# Autodesk Inventor assembly: Robot arm 01
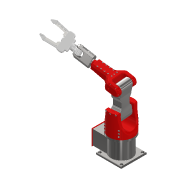
[picture p0: Inventor's stored thumbnail of the model, 180x180]
Saved by Autodesk Inventor 2020.3 (Build 243373010, 373A)
## iProperties
Created: 2021-04-17
Part Number: Robot arm 01
Document SubType Name: Assembly
Designer: marti
Mass: 362095 g
Surface Area: 35809.9 cm^2
Volume: 47437.3 cm^3
Density: 7.63313 g/cm^3
Author: marti
## Documents named in this file (30)
- C:\Users\marti\Documents\Inventor\RobotManipulateArm\17.4.2021 - Complete new IDEA\Robot arm 01.iam
- C:\Users\marti\Documents\Inventor\RobotManipulateArm\17.4.2021 - Complete new IDEA\Cover of robot - base upper part 02.ipt
- C:\Users\marti\Documents\Inventor\RobotManipulateArm\17.4.2021 - Complete new IDEA\Ground base of robot.ipt
- C:\Users\marti\Documents\Inventor\RobotManipulateArm\17.4.2021 - Complete new IDEA\base for robot 1\Base for robot 2.ipt
- C:\Users\marti\Documents\Inventor\RobotManipulateArm\17.4.2021 - Complete new IDEA\Servomotor_1.iam
- C:\Users\marti\Documents\Inventor\RobotManipulateArm\17.4.2021 - Complete new IDEA\Robot arm part 01.ipt
- C:\Users\marti\Documents\Inventor\RobotManipulateArm\17.4.2021 - Complete new IDEA\Head of robot arrm.ipt
- C:\Users\marti\Documents\Inventor\RobotManipulateArm\17.4.2021 - Complete new IDEA\Cover of robot base L.ipt
- C:\Users\marti\Documents\Inventor\Content Center Files\R2020\en-US\ISO 4762(1)\DIN EN ISO 4762 - M14 x 30.ipt
- C:\Users\marti\Documents\Inventor\RobotManipulateArm\17.4.2021 - Complete new IDEA\Cover of robot base R.ipt
- C:\Users\marti\Documents\Inventor\RobotManipulateArm\17.4.2021 - Complete new IDEA\Cover part of robot arm.ipt
- C:\Users\marti\Documents\Inventor\Content Center Files\R2020\en-US\ISO 4762(1)\DIN EN ISO 4762 - M10 x 25.ipt
- C:\Users\marti\Documents\Inventor\Content Center Files\R2020\en-US\ISO 4762(1)\DIN EN ISO 4762 - M12 x 25.ipt
- C:\Users\marti\Documents\Inventor\RobotManipulateArm\17.4.2021 - Complete new IDEA\Cover part of robot arm bottom side.ipt
- C:\Users\marti\Documents\Inventor\RobotManipulateArm\17.4.2021 - Complete new IDEA\Cover of base.ipt
- C:\Users\marti\Documents\Inventor\Content Center Files\R2020\en-US\ISO 4762(1)\DIN EN ISO 4762 - M10 x 16.ipt
- C:\Users\marti\Documents\Inventor\RobotManipulateArm\17.4.2021 - Complete new IDEA\Servo\Servo 250 W.iam
- C:\Users\marti\Documents\Inventor\RobotManipulateArm\17.4.2021 - Complete new IDEA\Cover for robot head.ipt
- C:\Users\marti\Documents\Inventor\RobotManipulateArm\17.4.2021 - Complete new IDEA\Upper cover of robot head.ipt
- C:\Users\marti\Documents\Inventor\Content Center Files\R2020\en-US\BS 4168(2)\BS 4168 - M4 x 20(2).ipt
- C:\Users\marti\Documents\Inventor\RobotManipulateArm\17.4.2021 - Complete new IDEA\Cover of robot upper base.ipt
- C:\Users\marti\Documents\Inventor\RobotManipulateArm\17.4.2021 - Complete new IDEA\Cover of robot- side part - base upper part 02.ipt
- C:\Users\marti\Documents\Inventor\RobotManipulateArm\17.4.2021 - Complete new IDEA\Cover of robot- side part - base upper part 01.ipt
- C:\Users\marti\Documents\Inventor\RobotManipulateArm\17.4.2021 - Complete new IDEA\Planetery gearbox.iam
- C:\Users\marti\Documents\Inventor\RobotManipulateArm\17.4.2021 - Complete new IDEA\Gearbox.iam
- C:\Users\marti\Documents\Inventor\RobotManipulateArm\17.4.2021 - Complete new IDEA\Tilting head.iam
- C:\Users\marti\Documents\Inventor\RobotManipulateArm\17.4.2021 - Complete new IDEA\Head belt gear.iam
- C:\Users\marti\Documents\Inventor\RobotManipulateArm\17.4.2021 - Complete new IDEA\Head belt gear 2.iam
- C:\Users\marti\Documents\Inventor\RobotManipulateArm\17.4.2021 - Complete new IDEA\Head gear shaft 2.iam
- C:\Users\marti\Documents\Inventor\RobotManipulateArm\17.4.2021 - Complete new IDEA\Gripper.iam
## Components (94 placed, 29 different names)
1. Cover of robot - base upper part 02:1 — Mate:7, Mate:10, Mate:11, Flush:3, Flush:4, Angle:1, Angle:2, Angle:3, Angle:4, Mate:71, Mate:184, Mate:185, Mate:186, Mate:187, Mate:189, Flush:26, Mate:190, Mate:191, Mate:194, Mate:195, Mate:196, Mate:198
2. Ground base of robot:1 — Mate:1, Mate:2, Mate:3, Mate:4, Mate:5, Mate:121, Mate:124, Mate:125, Mate:126, Mate:127, Mate:128, Mate:129, Mate:130, Mate:131, Mate:132, Mate:133, Mate:134, Mate:135, Mate:136, Mate:137, Mate:138, Mate:139, Mate:140, Mate:141, Mate:142, Mate:143, Mate:144, Mate:145, Mate:146, Mate:147
3. Base for robot 2:1 — Mate:4, Mate:5, Mate:7, Mate:30, Mate:31, Mate:33, Mate:40, Mate:41, Mate:43, Mate:44, Mate:52, Mate:53, Mate:54, Mate:59, Mate:61, Mate:194, Mate:197, Flush:27
4. Servomotor_1:5 [sub-assembly] — Mate:10, Flush:4, Mate:188
5. Servomotor_1:6 [sub-assembly] — Mate:11, Flush:3, Mate:72
6. Robot arm part 01:1 — Angle:2, Angle:4, Mate:71, Mate:72, Mate:73, Mate:74, Mate:75, Mate:78, Mate:79, Mate:80, Mate:81, Mate:82, Mate:84, Mate:85, Mate:87, Mate:88, Mate:89, Mate:90, Mate:91, Mate:92, Mate:93, Mate:94, Mate:95, Mate:96, Mate:97, Mate:98, Mate:99, Mate:100, Mate:101, Mate:102, Mate:103, Mate:104, Mate:105, Mate:107, Mate:108, Mate:109, Mate:110, Mate:111, Mate:112, Mate:113, Mate:114, Mate:115, Mate:116, Mate:117, Mate:118, Mate:148, Mate:149
7. Cover of robot base L:1 — Mate:30, Mate:31, Mate:33, Mate:34, Mate:35, Mate:36, Mate:37, Mate:38, Mate:39, Mate:42, Mate:45, Mate:46, Mate:47, Mate:48, Mate:49, Mate:50, Mate:51
8. DIN EN ISO 4762 M14 x 30:1 — Mate:55, Mate:56
9. DIN EN ISO 4762 M14 x 30:4 — Mate:34, Mate:35
10. DIN EN ISO 4762 M14 x 30:5 — Mate:36, Mate:37
11. DIN EN ISO 4762 M14 x 30:6 — Mate:38, Mate:39
12. DIN EN ISO 4762 M14 x 30:7 — Mate:40, Mate:47
13. DIN EN ISO 4762 M14 x 30:8 — Mate:42, Mate:49
14. DIN EN ISO 4762 M14 x 30:9 — Mate:43, Mate:46
15. DIN EN ISO 4762 M14 x 30:10 — Mate:44, Mate:45
16. DIN EN ISO 4762 M14 x 30:11 — Mate:41, Mate:48
17. DIN EN ISO 4762 M14 x 30:12 — Mate:50, Mate:51
18. Cover of robot base R:1 — Mate:52, Mate:53, Mate:54, Mate:55, Mate:56, Mate:57, Mate:58, Mate:60, Mate:62, Mate:63, Mate:64
19. DIN EN ISO 4762 M14 x 30:13 — Mate:57, Mate:58
20. DIN EN ISO 4762 M14 x 30:21 — Mate:63, Mate:64
21. Cover part of robot arm:2 — Mate:73, Mate:74, Mate:75, Mate:83
22. DIN EN ISO 4762 M10 x 25:17 — Mate:82, Mate:83
23. DIN EN ISO 4762 M10 x 25:18 — Mate:78, Mate:79
24. DIN EN ISO 4762 M10 x 25:19 — Mate:84, Mate:85
25. DIN EN ISO 4762 M10 x 25:21 — Mate:80, Mate:81
26. DIN EN ISO 4762 M10 x 25:22 — Mate:87, Mate:88
27. DIN EN ISO 4762 M10 x 25:23 — Mate:89, Mate:90
28. Cover part of robot arm:3 — Mate:91, Mate:92, Mate:93
29. DIN EN ISO 4762 M10 x 25:24 — Mate:98, Mate:99
30. DIN EN ISO 4762 M10 x 25:25 — Mate:94, Mate:95
31. DIN EN ISO 4762 M10 x 25:26 — Mate:104, Mate:105
32. DIN EN ISO 4762 M10 x 25:27 — Mate:96, Mate:97
33. DIN EN ISO 4762 M10 x 25:28 — Mate:100, Mate:101
34. DIN EN ISO 4762 M10 x 25:29 — Mate:102, Mate:103
35. Cover part of robot arm bottom side:1 — Mate:107, Mate:108, Mate:116, Mate:117, Mate:118
36. DIN EN ISO 4762 M12 x 25:3 — Mate:111, Mate:112, Mate:113
37. Cover of base:1 — Mate:121
38. DIN EN ISO 4762 M10 x 16:1 — Mate:124, Mate:125
39. DIN EN ISO 4762 M10 x 16:2 — Mate:126, Mate:127
40. DIN EN ISO 4762 M10 x 16:3 — Mate:128, Mate:129
41. DIN EN ISO 4762 M10 x 16:4 — Mate:130, Mate:131
42. DIN EN ISO 4762 M10 x 16:5 — Mate:132, Mate:133
43. DIN EN ISO 4762 M10 x 16:6 — Mate:134, Mate:135
44. DIN EN ISO 4762 M10 x 16:7 — Mate:136, Mate:137
45. DIN EN ISO 4762 M10 x 16:8 — Mate:138, Mate:139
46. DIN EN ISO 4762 M10 x 16:9 — Mate:140, Mate:141
47. DIN EN ISO 4762 M10 x 16:10 — Mate:142, Mate:143
48. DIN EN ISO 4762 M10 x 16:11 — Mate:144, Mate:145
49. DIN EN ISO 4762 M10 x 16:12 — Mate:146, Mate:147
50. Head of robot arrm:2 — Mate:148, Mate:149, Mate:150, Mate:151, Mate:152, Mate:153, Mate:154, Mate:155, Mate:156, Mate:157, Mate:158, Mate:159, Mate:161, Mate:162, Mate:163, Mate:164, Mate:165, Mate:166, Mate:167, Mate:168, Mate:169, Mate:170, Mate:183, Mate:200, Mate:203, Mate:204, Mate:206, Mate:208, Flush:29, Flush:31, Mate:210, Mate:212, Mate:213
51. Servo 250 W:2 [sub-assembly] — Mate:183, Mate:203, Mate:205, Flush:32
52. Cover for robot head:1 — Mate:150, Mate:151, Mate:152
53. Cover for robot head:2 — Mate:153, Mate:154, Mate:155, Mate:160
54. Upper cover of robot head:1 — Mate:156, Mate:157, Mate:158
55. BS 4168 : Part 2 Hexagon socket screws and wrench keys, metric series- Specification for hexagon set screws with flat point - Metric M4 x 20:1 — Mate:159, Mate:160, Flush:5, Flush:8, Flush:10
56. BS 4168 : Part 2 Hexagon socket screws and wrench keys, metric series- Specification for hexagon set screws with flat point - Metric M4 x 20:2 — Mate:162, Flush:6, Flush:13
57. BS 4168 : Part 2 Hexagon socket screws and wrench keys, metric series- Specification for hexagon set screws with flat point - Metric M4 x 20:3 — Mate:163, Flush:9, Flush:12
58. BS 4168 : Part 2 Hexagon socket screws and wrench keys, metric series- Specification for hexagon set screws with flat point - Metric M4 x 20:4 — Mate:164, Flush:8, Flush:9, Flush:11
59. BS 4168 : Part 2 Hexagon socket screws and wrench keys, metric series- Specification for hexagon set screws with flat point - Metric M4 x 20:5 — Mate:167, Flush:11
60. BS 4168 : Part 2 Hexagon socket screws and wrench keys, metric series- Specification for hexagon set screws with flat point - Metric M4 x 20:6 — Mate:166, Flush:10
61. BS 4168 : Part 2 Hexagon socket screws and wrench keys, metric series- Specification for hexagon set screws with flat point - Metric M4 x 20:7 — Mate:168, Flush:12
62. BS 4168 : Part 2 Hexagon socket screws and wrench keys, metric series- Specification for hexagon set screws with flat point - Metric M4 x 20:8 — Mate:169, Flush:13
63. BS 4168 : Part 2 Hexagon socket screws and wrench keys, metric series- Specification for hexagon set screws with flat point - Metric M4 x 20:9 — Mate:165, Flush:7
64. BS 4168 : Part 2 Hexagon socket screws and wrench keys, metric series- Specification for hexagon set screws with flat point - Metric M4 x 20:10 — Mate:161, Flush:5, Flush:6, Flush:7, Flush:14
65. BS 4168 : Part 2 Hexagon socket screws and wrench keys, metric series- Specification for hexagon set screws with flat point - Metric M4 x 20:11 — Mate:170, Flush:14
66. Cover of robot upper base:2 — Mate:184, Mate:185, Mate:186, Mate:192
67. Cover of robot- side part - base upper part 02:1 — Mate:187, Mate:188, Mate:189, Flush:26
68. Cover of robot- side part - base upper part 01:1 — Mate:190, Mate:191, Mate:192
69. Planetery gearbox:1 [sub-assembly] — Mate:195, Mate:196, Mate:199
70. Servomotor_1:7 [sub-assembly] — Mate:198, Mate:199
71. Gearbox:1 [sub-assembly] — Mate:197, Flush:27
72. Tilting head:1 [sub-assembly] — Mate:200, Mate:202, Rotation:1, Mate:213, Mate:214, Mate:215, Mate:216
73. Servo 250 W:3 [sub-assembly] — Mate:204, Mate:205, Flush:30
74. Head belt gear:1 [sub-assembly] — Mate:209, Flush:31, Mate:210, Flush:32, Flush:34
75. Head belt gear 2:1 [sub-assembly] — Mate:206, Mate:207, Mate:208, Flush:29, Flush:30, Mate:211, Flush:33
76. Head gear shaft 2:1 [sub-assembly] — Mate:212, Flush:34
77. Head gear shaft 2:2 [sub-assembly] — Mate:211, Flush:33, Rotation:1
78. Gripper:1 [sub-assembly] — Mate:214, Mate:215, Mate:216
79. DIN EN ISO 4762 M14 x 30:15 — Mate:59, Mate:60
80. DIN EN ISO 4762 M14 x 30:16 — Mate:61, Mate:62
81. DIN EN ISO 4762 M14 x 30:17
82. DIN EN ISO 4762 M14 x 30:18
83. DIN EN ISO 4762 M14 x 30:19
84. DIN EN ISO 4762 M14 x 30:20
85. DIN EN ISO 4762 M12 x 25:1 — Mate:109, Mate:110
86. DIN EN ISO 4762 M12 x 25:2 — Mate:114, Mate:115
87. DIN EN ISO 4762 M12 x 25:4
88. DIN EN ISO 4762 M12 x 25:5
89. DIN EN ISO 4762 M12 x 25:6
90. DIN EN ISO 4762 M12 x 25:7
91. DIN EN ISO 4762 M12 x 25:8
92. DIN EN ISO 4762 M12 x 25:9
93. DIN EN ISO 4762 M12 x 25:10
94. DIN EN ISO 4762 M12 x 25:11
## Component patterns: (3 elements, first: DIN EN ISO 4762 M14 x 30:15 + DIN EN ISO 4762 M14 x 30:16), (5 elements, first: DIN EN ISO 4762 M12 x 25:1 + DIN EN ISO 4762 M12 x 25:2)
## Relationships (191: Mate 166, Flush 20, Angle 4, RelateRotation 1)
- Mate:1: Ground base of robot:1
- Mate:2: Ground base of robot:1
- Mate:3: Ground base of robot:1
- Mate:4: Ground base of robot:1 ↔ Base for robot 2:1
- Mate:5: Ground base of robot:1 ↔ Base for robot 2:1
- Mate:7 (8.5 mm): Cover of robot - base upper part 02:1 ↔ Base for robot 2:1
- Mate:10: Cover of robot - base upper part 02:1 ↔ Servomotor_1:5
- Mate:11: Cover of robot - base upper part 02:1 ↔ Servomotor_1:6
- Flush:3: Cover of robot - base upper part 02:1 ↔ Servomotor_1:6
- Flush:4: Cover of robot - base upper part 02:1 ↔ Servomotor_1:5
- Mate:30: Base for robot 2:1 ↔ Cover of robot base L:1
- Mate:31: Base for robot 2:1 ↔ Cover of robot base L:1
- Mate:33: Base for robot 2:1 ↔ Cover of robot base L:1
- Mate:34: Cover of robot base L:1 ↔ DIN EN ISO 4762 M14 x 30:4
- Mate:35: Cover of robot base L:1 ↔ DIN EN ISO 4762 M14 x 30:4
- Mate:36: Cover of robot base L:1 ↔ DIN EN ISO 4762 M14 x 30:5
- Mate:37: Cover of robot base L:1 ↔ DIN EN ISO 4762 M14 x 30:5
- Mate:38: Cover of robot base L:1 ↔ DIN EN ISO 4762 M14 x 30:6
- Mate:39: Cover of robot base L:1 ↔ DIN EN ISO 4762 M14 x 30:6
- Mate:40: Base for robot 2:1 ↔ DIN EN ISO 4762 M14 x 30:7
- Mate:41: Base for robot 2:1 ↔ DIN EN ISO 4762 M14 x 30:11
- Mate:42: Cover of robot base L:1 ↔ DIN EN ISO 4762 M14 x 30:8
- Mate:43: Base for robot 2:1 ↔ DIN EN ISO 4762 M14 x 30:9
- Mate:44: Base for robot 2:1 ↔ DIN EN ISO 4762 M14 x 30:10
- Mate:45: Cover of robot base L:1 ↔ DIN EN ISO 4762 M14 x 30:10
- Mate:46: Cover of robot base L:1 ↔ DIN EN ISO 4762 M14 x 30:9
- Mate:47: Cover of robot base L:1 ↔ DIN EN ISO 4762 M14 x 30:7
- Mate:48: Cover of robot base L:1 ↔ DIN EN ISO 4762 M14 x 30:11
- Mate:49: Cover of robot base L:1 ↔ DIN EN ISO 4762 M14 x 30:8
- Mate:50: Cover of robot base L:1 ↔ DIN EN ISO 4762 M14 x 30:12
- Mate:51: Cover of robot base L:1 ↔ DIN EN ISO 4762 M14 x 30:12
- Mate:52: Base for robot 2:1 ↔ Cover of robot base R:1
- Mate:53: Base for robot 2:1 ↔ Cover of robot base R:1
- Mate:54: Base for robot 2:1 ↔ Cover of robot base R:1
- Mate:55: DIN EN ISO 4762 M14 x 30:1 ↔ Cover of robot base R:1
- Mate:56: DIN EN ISO 4762 M14 x 30:1 ↔ Cover of robot base R:1
- Mate:57: Cover of robot base R:1 ↔ DIN EN ISO 4762 M14 x 30:13
- Mate:58: Cover of robot base R:1 ↔ DIN EN ISO 4762 M14 x 30:13
- Mate:59: Base for robot 2:1 ↔ DIN EN ISO 4762 M14 x 30:15
- Mate:60: Cover of robot base R:1 ↔ DIN EN ISO 4762 M14 x 30:15
- Angle:1 (0 deg): Cover of robot - base upper part 02:1
- Mate:61: Base for robot 2:1 ↔ DIN EN ISO 4762 M14 x 30:16
- Mate:62: Cover of robot base R:1 ↔ DIN EN ISO 4762 M14 x 30:16
- Mate:63: Cover of robot base R:1 ↔ DIN EN ISO 4762 M14 x 30:21
- Mate:64: Cover of robot base R:1 ↔ DIN EN ISO 4762 M14 x 30:21
- Angle:2 (170 deg): Cover of robot - base upper part 02:1 ↔ Robot arm part 01:1
- Angle:3 (175 deg): Cover of robot - base upper part 02:1
- Angle:4 (75 deg): Cover of robot - base upper part 02:1 ↔ Robot arm part 01:1
- Mate:71 (2 mm): Cover of robot - base upper part 02:1 ↔ Robot arm part 01:1
- Mate:72: Servomotor_1:6 ↔ Robot arm part 01:1
- Mate:73: Robot arm part 01:1 ↔ Cover part of robot arm:2
- Mate:74: Robot arm part 01:1 ↔ Cover part of robot arm:2
- Mate:75: Robot arm part 01:1 ↔ Cover part of robot arm:2
- Mate:78: Robot arm part 01:1 ↔ DIN EN ISO 4762 M10 x 25:18
- Mate:79: Robot arm part 01:1 ↔ DIN EN ISO 4762 M10 x 25:18
- Mate:80: Robot arm part 01:1 ↔ DIN EN ISO 4762 M10 x 25:21
- Mate:81: Robot arm part 01:1 ↔ DIN EN ISO 4762 M10 x 25:21
- Mate:82: Robot arm part 01:1 ↔ DIN EN ISO 4762 M10 x 25:17
- Mate:83: Cover part of robot arm:2 ↔ DIN EN ISO 4762 M10 x 25:17
- Mate:84: Robot arm part 01:1 ↔ DIN EN ISO 4762 M10 x 25:19
- Mate:85: Robot arm part 01:1 ↔ DIN EN ISO 4762 M10 x 25:19
- Mate:87: Robot arm part 01:1 ↔ DIN EN ISO 4762 M10 x 25:22
- Mate:88: Robot arm part 01:1 ↔ DIN EN ISO 4762 M10 x 25:22
- Mate:89: Robot arm part 01:1 ↔ DIN EN ISO 4762 M10 x 25:23
- Mate:90: Robot arm part 01:1 ↔ DIN EN ISO 4762 M10 x 25:23
- Mate:91: Robot arm part 01:1 ↔ Cover part of robot arm:3
- Mate:92: Robot arm part 01:1 ↔ Cover part of robot arm:3
- Mate:93: Robot arm part 01:1 ↔ Cover part of robot arm:3
- Mate:94: Robot arm part 01:1 ↔ DIN EN ISO 4762 M10 x 25:25
- Mate:95: Robot arm part 01:1 ↔ DIN EN ISO 4762 M10 x 25:25
- Mate:96: Robot arm part 01:1 ↔ DIN EN ISO 4762 M10 x 25:27
- Mate:97: Robot arm part 01:1 ↔ DIN EN ISO 4762 M10 x 25:27
- Mate:98: Robot arm part 01:1 ↔ DIN EN ISO 4762 M10 x 25:24
- Mate:99: Robot arm part 01:1 ↔ DIN EN ISO 4762 M10 x 25:24
- Mate:100: Robot arm part 01:1 ↔ DIN EN ISO 4762 M10 x 25:28
- Mate:101: Robot arm part 01:1 ↔ DIN EN ISO 4762 M10 x 25:28
- Mate:102: Robot arm part 01:1 ↔ DIN EN ISO 4762 M10 x 25:29
- Mate:103: Robot arm part 01:1 ↔ DIN EN ISO 4762 M10 x 25:29
- Mate:104: Robot arm part 01:1 ↔ DIN EN ISO 4762 M10 x 25:26
- Mate:105: Robot arm part 01:1 ↔ DIN EN ISO 4762 M10 x 25:26
- Mate:107: Robot arm part 01:1 ↔ Cover part of robot arm bottom side:1
- Mate:108: Robot arm part 01:1 ↔ Cover part of robot arm bottom side:1
- Mate:109: Robot arm part 01:1 ↔ DIN EN ISO 4762 M12 x 25:1
- Mate:110: Robot arm part 01:1 ↔ DIN EN ISO 4762 M12 x 25:1
- Mate:111: Robot arm part 01:1 ↔ DIN EN ISO 4762 M12 x 25:3
- Mate:112: Robot arm part 01:1 ↔ DIN EN ISO 4762 M12 x 25:3
- Mate:113: Robot arm part 01:1 ↔ DIN EN ISO 4762 M12 x 25:3
- Mate:114: Robot arm part 01:1 ↔ DIN EN ISO 4762 M12 x 25:2
- Mate:115: Robot arm part 01:1 ↔ DIN EN ISO 4762 M12 x 25:2
- Mate:116: Robot arm part 01:1 ↔ Cover part of robot arm bottom side:1
- Mate:117: Robot arm part 01:1 ↔ Cover part of robot arm bottom side:1
- Mate:118: Robot arm part 01:1 ↔ Cover part of robot arm bottom side:1
- Mate:121: Ground base of robot:1 ↔ Cover of base:1
- Mate:124: Ground base of robot:1 ↔ DIN EN ISO 4762 M10 x 16:1
- Mate:125: Ground base of robot:1 ↔ DIN EN ISO 4762 M10 x 16:1
- Mate:126: Ground base of robot:1 ↔ DIN EN ISO 4762 M10 x 16:2
- Mate:127: Ground base of robot:1 ↔ DIN EN ISO 4762 M10 x 16:2
- Mate:128: Ground base of robot:1 ↔ DIN EN ISO 4762 M10 x 16:3
- Mate:129: Ground base of robot:1 ↔ DIN EN ISO 4762 M10 x 16:3
- Mate:130: Ground base of robot:1 ↔ DIN EN ISO 4762 M10 x 16:4
- Mate:131: Ground base of robot:1 ↔ DIN EN ISO 4762 M10 x 16:4
- Mate:132: Ground base of robot:1 ↔ DIN EN ISO 4762 M10 x 16:5
- Mate:133: Ground base of robot:1 ↔ DIN EN ISO 4762 M10 x 16:5
- Mate:134: Ground base of robot:1 ↔ DIN EN ISO 4762 M10 x 16:6
- Mate:135: Ground base of robot:1 ↔ DIN EN ISO 4762 M10 x 16:6
- Mate:136: Ground base of robot:1 ↔ DIN EN ISO 4762 M10 x 16:7
- Mate:137: Ground base of robot:1 ↔ DIN EN ISO 4762 M10 x 16:7
- Mate:138: Ground base of robot:1 ↔ DIN EN ISO 4762 M10 x 16:8
- Mate:139: Ground base of robot:1 ↔ DIN EN ISO 4762 M10 x 16:8
- Mate:140: Ground base of robot:1 ↔ DIN EN ISO 4762 M10 x 16:9
- Mate:141: Ground base of robot:1 ↔ DIN EN ISO 4762 M10 x 16:9
- Mate:142: Ground base of robot:1 ↔ DIN EN ISO 4762 M10 x 16:10
- Mate:143: Ground base of robot:1 ↔ DIN EN ISO 4762 M10 x 16:10
- Mate:144: Ground base of robot:1 ↔ DIN EN ISO 4762 M10 x 16:11
- Mate:145: Ground base of robot:1 ↔ DIN EN ISO 4762 M10 x 16:11
- Mate:146: Ground base of robot:1 ↔ DIN EN ISO 4762 M10 x 16:12
- Mate:147: Ground base of robot:1 ↔ DIN EN ISO 4762 M10 x 16:12
- Mate:148: Robot arm part 01:1 ↔ Head of robot arrm:2
- Mate:149: Robot arm part 01:1 ↔ Head of robot arrm:2
- Mate:150: Head of robot arrm:2 ↔ Cover for robot head:1
- Mate:151: Head of robot arrm:2 ↔ Cover for robot head:1
- Mate:152: Head of robot arrm:2 ↔ Cover for robot head:1
- Mate:153: Head of robot arrm:2 ↔ Cover for robot head:2
- Mate:154: Head of robot arrm:2 ↔ Cover for robot head:2
- Mate:155: Head of robot arrm:2 ↔ Cover for robot head:2
- Mate:156: Head of robot arrm:2 ↔ Upper cover of robot head:1
- Mate:157: Head of robot arrm:2 ↔ Upper cover of robot head:1
- Mate:158: Head of robot arrm:2 ↔ Upper cover of robot head:1
- Mate:159: Head of robot arrm:2 ↔ BS 4168 : Part 2 Hexagon socket screws and wrench keys, metric series- Specification for hexagon set screws with flat point - Metric M4 x 20:1
- Mate:160: Cover for robot head:2 ↔ BS 4168 : Part 2 Hexagon socket screws and wrench keys, metric series- Specification for hexagon set screws with flat point - Metric M4 x 20:1
- Mate:161: Head of robot arrm:2 ↔ BS 4168 : Part 2 Hexagon socket screws and wrench keys, metric series- Specification for hexagon set screws with flat point - Metric M4 x 20:10
- Flush:5: BS 4168 : Part 2 Hexagon socket screws and wrench keys, metric series- Specification for hexagon set screws with flat point - Metric M4 x 20:1 ↔ BS 4168 : Part 2 Hexagon socket screws and wrench keys, metric series- Specification for hexagon set screws with flat point - Metric M4 x 20:10
- Mate:162: Head of robot arrm:2 ↔ BS 4168 : Part 2 Hexagon socket screws and wrench keys, metric series- Specification for hexagon set screws with flat point - Metric M4 x 20:2
- Flush:6: BS 4168 : Part 2 Hexagon socket screws and wrench keys, metric series- Specification for hexagon set screws with flat point - Metric M4 x 20:2 ↔ BS 4168 : Part 2 Hexagon socket screws and wrench keys, metric series- Specification for hexagon set screws with flat point - Metric M4 x 20:10
- Mate:163: Head of robot arrm:2 ↔ BS 4168 : Part 2 Hexagon socket screws and wrench keys, metric series- Specification for hexagon set screws with flat point - Metric M4 x 20:3
- Mate:164: Head of robot arrm:2 ↔ BS 4168 : Part 2 Hexagon socket screws and wrench keys, metric series- Specification for hexagon set screws with flat point - Metric M4 x 20:4
- Mate:165: Head of robot arrm:2 ↔ BS 4168 : Part 2 Hexagon socket screws and wrench keys, metric series- Specification for hexagon set screws with flat point - Metric M4 x 20:9
- Flush:7: BS 4168 : Part 2 Hexagon socket screws and wrench keys, metric series- Specification for hexagon set screws with flat point - Metric M4 x 20:9 ↔ BS 4168 : Part 2 Hexagon socket screws and wrench keys, metric series- Specification for hexagon set screws with flat point - Metric M4 x 20:10
- Flush:8: BS 4168 : Part 2 Hexagon socket screws and wrench keys, metric series- Specification for hexagon set screws with flat point - Metric M4 x 20:1 ↔ BS 4168 : Part 2 Hexagon socket screws and wrench keys, metric series- Specification for hexagon set screws with flat point - Metric M4 x 20:4
- Flush:9: BS 4168 : Part 2 Hexagon socket screws and wrench keys, metric series- Specification for hexagon set screws with flat point - Metric M4 x 20:3 ↔ BS 4168 : Part 2 Hexagon socket screws and wrench keys, metric series- Specification for hexagon set screws with flat point - Metric M4 x 20:4
- Mate:166: Head of robot arrm:2 ↔ BS 4168 : Part 2 Hexagon socket screws and wrench keys, metric series- Specification for hexagon set screws with flat point - Metric M4 x 20:6
- Flush:10: BS 4168 : Part 2 Hexagon socket screws and wrench keys, metric series- Specification for hexagon set screws with flat point - Metric M4 x 20:1 ↔ BS 4168 : Part 2 Hexagon socket screws and wrench keys, metric series- Specification for hexagon set screws with flat point - Metric M4 x 20:6
- Mate:167: Head of robot arrm:2 ↔ BS 4168 : Part 2 Hexagon socket screws and wrench keys, metric series- Specification for hexagon set screws with flat point - Metric M4 x 20:5
- Flush:11: BS 4168 : Part 2 Hexagon socket screws and wrench keys, metric series- Specification for hexagon set screws with flat point - Metric M4 x 20:4 ↔ BS 4168 : Part 2 Hexagon socket screws and wrench keys, metric series- Specification for hexagon set screws with flat point - Metric M4 x 20:5
- Mate:168: Head of robot arrm:2 ↔ BS 4168 : Part 2 Hexagon socket screws and wrench keys, metric series- Specification for hexagon set screws with flat point - Metric M4 x 20:7
- Flush:12: BS 4168 : Part 2 Hexagon socket screws and wrench keys, metric series- Specification for hexagon set screws with flat point - Metric M4 x 20:3 ↔ BS 4168 : Part 2 Hexagon socket screws and wrench keys, metric series- Specification for hexagon set screws with flat point - Metric M4 x 20:7
- Mate:169: Head of robot arrm:2 ↔ BS 4168 : Part 2 Hexagon socket screws and wrench keys, metric series- Specification for hexagon set screws with flat point - Metric M4 x 20:8
- Flush:13: BS 4168 : Part 2 Hexagon socket screws and wrench keys, metric series- Specification for hexagon set screws with flat point - Metric M4 x 20:2 ↔ BS 4168 : Part 2 Hexagon socket screws and wrench keys, metric series- Specification for hexagon set screws with flat point - Metric M4 x 20:8
- Mate:170: Head of robot arrm:2 ↔ BS 4168 : Part 2 Hexagon socket screws and wrench keys, metric series- Specification for hexagon set screws with flat point - Metric M4 x 20:11
- Flush:14: BS 4168 : Part 2 Hexagon socket screws and wrench keys, metric series- Specification for hexagon set screws with flat point - Metric M4 x 20:10 ↔ BS 4168 : Part 2 Hexagon socket screws and wrench keys, metric series- Specification for hexagon set screws with flat point - Metric M4 x 20:11
- Mate:183: Head of robot arrm:2 ↔ Servo 250 W:2
- Mate:184: Cover of robot - base upper part 02:1 ↔ Cover of robot upper base:2
- Mate:185: Cover of robot - base upper part 02:1 ↔ Cover of robot upper base:2
- Mate:186: Cover of robot - base upper part 02:1 ↔ Cover of robot upper base:2
- Mate:187: Cover of robot - base upper part 02:1 ↔ Cover of robot- side part - base upper part 02:1
- Mate:188: Servomotor_1:5 ↔ Cover of robot- side part - base upper part 02:1
- Mate:189: Cover of robot - base upper part 02:1 ↔ Cover of robot- side part - base upper part 02:1
- Flush:26: Cover of robot - base upper part 02:1 ↔ Cover of robot- side part - base upper part 02:1
- Mate:190: Cover of robot - base upper part 02:1 ↔ Cover of robot- side part - base upper part 01:1
- Mate:191: Cover of robot - base upper part 02:1 ↔ Cover of robot- side part - base upper part 01:1
- Mate:192: Cover of robot upper base:2 ↔ Cover of robot- side part - base upper part 01:1
- Mate:194: Cover of robot - base upper part 02:1 ↔ Base for robot 2:1
- Mate:195: Cover of robot - base upper part 02:1 ↔ Planetery gearbox:1
- Mate:196: Cover of robot - base upper part 02:1 ↔ Planetery gearbox:1
- Mate:197: Base for robot 2:1 ↔ Gearbox:1
- Flush:27: Base for robot 2:1 ↔ Gearbox:1
- Mate:198: Cover of robot - base upper part 02:1 ↔ Servomotor_1:7
- Mate:199: Planetery gearbox:1 ↔ Servomotor_1:7
- Mate:200: Head of robot arrm:2 ↔ Tilting head:1
- Mate:202: Tilting head:1
- Mate:203: Head of robot arrm:2 ↔ Servo 250 W:2
- Mate:204: Head of robot arrm:2 ↔ Servo 250 W:3
- Mate:205: Servo 250 W:2 ↔ Servo 250 W:3
- Mate:206: Head of robot arrm:2 ↔ Head belt gear 2:1
- Mate:207: Head belt gear 2:1
- Mate:208: Head of robot arrm:2 ↔ Head belt gear 2:1
- Flush:29 (2 mm): Head of robot arrm:2 ↔ Head belt gear 2:1
- Flush:30: Servo 250 W:3 ↔ Head belt gear 2:1
- Mate:209: Head belt gear:1
- Flush:31 (2 mm): Head of robot arrm:2 ↔ Head belt gear:1
- Mate:210: Head of robot arrm:2 ↔ Head belt gear:1
- Flush:32: Servo 250 W:2 ↔ Head belt gear:1
- Mate:211: Head belt gear 2:1 ↔ Head gear shaft 2:2
- Flush:33: Head belt gear 2:1 ↔ Head gear shaft 2:2
- Mate:212: Head of robot arrm:2 ↔ Head gear shaft 2:1
- Flush:34: Head belt gear:1 ↔ Head gear shaft 2:1
- Rotation:1 [RelateRotation] (1 ul): Tilting head:1 ↔ Head gear shaft 2:2
- Mate:213: Head of robot arrm:2 ↔ Tilting head:1
- Mate:214: Tilting head:1 ↔ Gripper:1
- Mate:215: Tilting head:1 ↔ Gripper:1
- Mate:216: Tilting head:1 ↔ Gripper:1
